# Autodesk Inventor assembly: Payload_Assembly
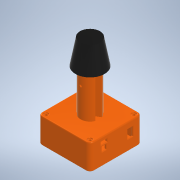
[picture p0: Inventor's stored thumbnail of the model, 180x180]
Saved by Autodesk Inventor 2020 (Build 240168000, 168)
## iProperties
Created: 2019-09-16
Part Number: Payload_Assembly
Document SubType Name: Assembly
Designer: jcocker
Author: jcocker
## Documents named in this file (4)
- \\engrfs904v\VCL.userspace\jcocker\Documents\Payload Data Acquisition\Arduino_Case\Payload_Assembly.iam
- \\engrfs904v\VCL.userspace\jcocker\Documents\Payload Data Acquisition\Arduino_Case\Arduino_case_bottom_JC_Rev2.ipt
- \\engrfs904v\VCL.userspace\jcocker\Documents\Payload Data Acquisition\Arduino_Case\Arduino_case_top_JC_Rev1.ipt
- \\engrfs904v\VCL.userspace\jcocker\Documents\Payload Data Acquisition\Arduino_Case\IP_Cap_JC.ipt
## Components (3 placed, 3 different names)
1. Arduino_case_bottom_JC_Rev2:1 — Flush:1, Mate:1, Flush:2
2. Arduino_case_top_JC_Rev1:1 — Flush:1, Mate:1, Flush:2, Mate:2, Mate:3
3. IP_Cap_JC:1 — Mate:2, Mate:3
## Relationships (5: Mate 3, Flush 2)
- Flush:1: Arduino_case_bottom_JC_Rev2:1 ↔ Arduino_case_top_JC_Rev1:1
- Mate:1: Arduino_case_bottom_JC_Rev2:1 ↔ Arduino_case_top_JC_Rev1:1
- Flush:2: Arduino_case_bottom_JC_Rev2:1 ↔ Arduino_case_top_JC_Rev1:1
- Mate:2: Arduino_case_top_JC_Rev1:1 ↔ IP_Cap_JC:1
- Mate:3: Arduino_case_top_JC_Rev1:1 ↔ IP_Cap_JC:1
